# Autodesk Inventor assembly: 000 ASY GBK Gubkinskiy
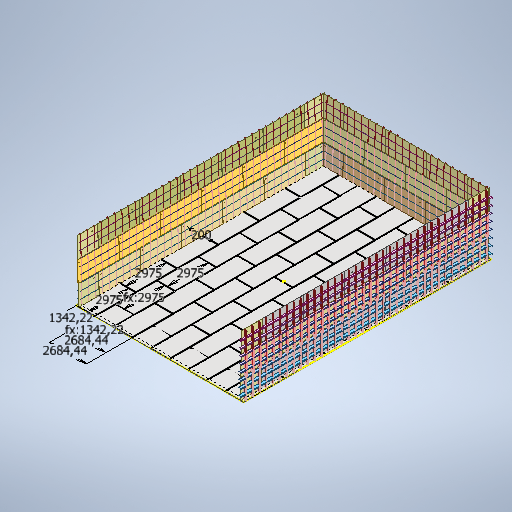
[picture p0: Inventor's stored thumbnail of the model, 512x512]
Saved by Autodesk Inventor 2026.2 (Build 302298000, 298)
## iProperties
Created: 2026-04-17
Part Number: 000 ASY GBK Gubkinskiy
Document SubType Name: Assembly
Designer: admin
Mass: 2.02017e+07 g
Surface Area: 1.30705e+07 cm^2
Volume: 2.57346e+06 cm^3
Density: 7.85 g/cm^3
Author: admin
## Documents named in this file (11)
- C:\Users\admin\Documents\Inventor\GBK-Gubkinskiy\000 ASY GBK Gubkinskiy.iam
- C:\Users\admin\Documents\Inventor\GBK-Gubkinskiy\GBK bottom.ipt
- C:\Users\admin\Documents\Inventor\GBK-Gubkinskiy\GBK dummy wall 1.ipt
- C:\Users\admin\Documents\Inventor\GBK-Gubkinskiy\GBK dummy wall 4.ipt
- C:\Users\admin\Documents\Inventor\GBK-Gubkinskiy\GBK overall model.ipt
- C:\Users\admin\Documents\Inventor\GBK-Gubkinskiy\ASY GBK 3110 wall shield Center 1.iam
- C:\Users\admin\Documents\Inventor\GBK-Gubkinskiy\ASY GBK 3210 wall shield Center 3.iam
- C:\Users\admin\Documents\Inventor\GBK-Gubkinskiy\ASY GBK 3310 wall shield Center 4.iam
- C:\Users\admin\Documents\Inventor\GBK-Gubkinskiy\ASY GBK длинная стенка.iam
- C:\Users\admin\Documents\Inventor\GBK-Gubkinskiy\090 ASY bottom.iam
- C:\Users\admin\Documents\Inventor\GBK-Gubkinskiy\ASY GBK короткая стенка.iam
## Components (12 placed, 10 different names)
1. GBK bottom.ipt:1 — Mate:10, Mate:11, Mate:12, Mate:13, Mate:14, Rigid:1, Flush:6, Flush:7, Flush:8, Flush:9, Flush:11, Flush:13
2. GBK dummy wall 1.ipt:1 — Mate:10
3. GBK dummy wall 1.ipt:2 — Mate:11, Mate:12
4. GBK dummy wall 4.ipt:1 — Mate:13, Mate:14
5. GBK overall model.ipt:1 — Rigid:1
6. ASY GBK длинная стенка.iam:1 [sub-assembly] — Flush:11
7. ASY GBK длинная стенка.iam:2 [sub-assembly] — Flush:5, Flush:6, Flush:9, Flush:12
8. ASY GBK 3210 wall shield Center 3.iam:1 [sub-assembly] — Rigid:2, Rigid:3
9. ASY GBK 3310 wall shield Center 4.iam:1 [sub-assembly] — Rigid:3
10. ASY GBK 3110 wall shield Center 1.iam:1 [sub-assembly] — Rigid:2, Mate:18, Flush:7
11. 090 ASY bottom.iam:1 [sub-assembly] — Mate:19, Flush:8
12. ASY GBK короткая стенка.iam:1 [sub-assembly] — Flush:12, Flush:13, Mate:20
## Relationships (21: Flush 9, Mate 9, WeldJoint 3)
- [Flush]: GBK bottom.ipt:1 ↔ ASY GBK длинная стенка.iam:1
- [Mate]: GBK bottom.ipt:1 ↔ ASY GBK длинная стенка.iam:1
- Mate:10: GBK bottom.ipt:1 ↔ GBK dummy wall 1.ipt:1
- Mate:11: GBK bottom.ipt:1 ↔ GBK dummy wall 1.ipt:2
- Mate:12: GBK bottom.ipt:1 ↔ GBK dummy wall 1.ipt:2
- Mate:13: GBK bottom.ipt:1 ↔ GBK dummy wall 4.ipt:1
- Mate:14: GBK bottom.ipt:1 ↔ GBK dummy wall 4.ipt:1
- Rigid:1 [WeldJoint]: GBK bottom.ipt:1 ↔ GBK overall model.ipt:1
- Flush:5: ASY GBK длинная стенка.iam:2
- Flush:6: GBK bottom.ipt:1 ↔ ASY GBK длинная стенка.iam:2
- Rigid:2 [WeldJoint]: ASY GBK 3210 wall shield Center 3.iam:1 ↔ ASY GBK 3110 wall shield Center 1.iam:1
- Rigid:3 [WeldJoint]: ASY GBK 3210 wall shield Center 3.iam:1 ↔ ASY GBK 3310 wall shield Center 4.iam:1
- Mate:18: ASY GBK 3110 wall shield Center 1.iam:1
- Flush:7: GBK bottom.ipt:1 ↔ ASY GBK 3110 wall shield Center 1.iam:1
- Mate:19: 090 ASY bottom.iam:1
- Flush:8: GBK bottom.ipt:1 ↔ 090 ASY bottom.iam:1
- Flush:9: GBK bottom.ipt:1 ↔ ASY GBK длинная стенка.iam:2
- Flush:11: GBK bottom.ipt:1 ↔ ASY GBK длинная стенка.iam:1
- Flush:12 (262 mm): ASY GBK длинная стенка.iam:2 ↔ ASY GBK короткая стенка.iam:1
- Flush:13: GBK bottom.ipt:1 ↔ ASY GBK короткая стенка.iam:1
- Mate:20: ASY GBK короткая стенка.iam:1
## Named parameters: Зазор_по_горизонту = 1 mm, d120_Зазор_по_горизонту = 1 mm, d141_Зазор_по_горизонту = 1 mm, d159_d141_Зазор_по_горизонту = 1 mm, d175_d141_Зазор_по_горизонту = 1 mm
